# Autodesk Inventor assembly: 組合3
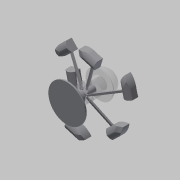
[picture p0: Inventor's stored thumbnail of the model, 180x180]
Saved by Autodesk Inventor 2018 (Build 220112000, 112)
## iProperties
Created: 2021-03-14
Part Number: 組合3
Material: 一般
Document SubType Name: Assembly
Designer: 王鼎鈞
Author: 王鼎鈞
## Documents named in this file (5)
- D:\2021顏家民\兩人組圖檔\組合3.iam
- D:\2021顏家民\兩人組圖檔\主體.ipt
- D:\2021顏家民\兩人組圖檔\底座構想3.ipt
- D:\2021顏家民\兩人組圖檔\支架3.ipt
- D:\2021顏家民\兩人組圖檔\容器.ipt
## Components (14 placed, 4 different names)
1. 主體:1 — 插入:1, 插入:2, 插入:3, 插入:4, 插入:5, 插入:6, 插入:7, 旋轉:1
2. 底座構想3:1 — 插入:1, 相切:1, 相切:2, 相切:3, 相切:4, 相切:5, 相切:6, 相切:7, 旋轉:1, 角度:1, 角度:2, 角度:3, 角度:4, 角度:5, 角度:6
3. 支架3:1 — 插入:2, 相切:1, 相切:6, 插入:12
4. 支架3:2 — 插入:3, 相切:5, 插入:11
5. 支架3:3 — 插入:5, 相切:3, 插入:8
6. 支架3:4 — 插入:4, 相切:4, 插入:9
7. 支架3:5 — 插入:7, 相切:7, 插入:13
8. 支架3:6 — 插入:6, 相切:2, 插入:10
9. 容器:1 — 插入:10, 角度:3
10. 容器:2 — 插入:11, 角度:4
11. 容器:3 — 插入:12, 角度:5
12. 容器:4 — 插入:8, 角度:1
13. 容器:5 — 插入:9, 角度:2
14. 容器:6 — 插入:13, 角度:6
## Relationships (27: Insert 13, Tangent 7, Angle 6, RevoluteJoint 1)
- 插入:1 [Insert]: 主體:1 ↔ 底座構想3:1
- 插入:2 [Insert]: 主體:1 ↔ 支架3:1
- 相切:1 [Tangent]: 底座構想3:1 ↔ 支架3:1
- 插入:3 [Insert]: 主體:1 ↔ 支架3:2
- 插入:4 [Insert]: 主體:1 ↔ 支架3:4
- 插入:5 [Insert]: 主體:1 ↔ 支架3:3
- 插入:6 [Insert]: 主體:1 ↔ 支架3:6
- 插入:7 [Insert]: 主體:1 ↔ 支架3:5
- 相切:2 [Tangent]: 底座構想3:1 ↔ 支架3:6
- 相切:3 [Tangent]: 底座構想3:1 ↔ 支架3:3
- 相切:4 [Tangent]: 底座構想3:1 ↔ 支架3:4
- 相切:5 [Tangent]: 底座構想3:1 ↔ 支架3:2
- 相切:6 [Tangent]: 底座構想3:1 ↔ 支架3:1
- 相切:7 [Tangent]: 底座構想3:1 ↔ 支架3:5
- 旋轉:1 [RevoluteJoint]: 主體:1 ↔ 底座構想3:1
- 插入:8 [Insert]: 支架3:3 ↔ 容器:4
- 角度:1 [Angle] (0 deg): 底座構想3:1 ↔ 容器:4
- 插入:9 [Insert]: 支架3:4 ↔ 容器:5
- 角度:2 [Angle] (0 deg): 底座構想3:1 ↔ 容器:5
- 插入:10 [Insert]: 支架3:6 ↔ 容器:1
- 角度:3 [Angle] (0 deg): 底座構想3:1 ↔ 容器:1
- 插入:11 [Insert]: 支架3:2 ↔ 容器:2
- 角度:4 [Angle] (0 deg): 底座構想3:1 ↔ 容器:2
- 插入:12 [Insert]: 支架3:1 ↔ 容器:3
- 角度:5 [Angle] (0 deg): 底座構想3:1 ↔ 容器:3
- 插入:13 [Insert]: 支架3:5 ↔ 容器:6
- 角度:6 [Angle] (0 deg): 底座構想3:1 ↔ 容器:6
